# Autodesk Inventor assembly: 8 ball mechanism 3
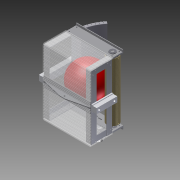
[picture p0: Inventor's stored thumbnail of the model, 180x180]
Saved by Autodesk Inventor 2012 (Build 160160000, 160)
## iProperties
Created: 2013-10-10
Part Number: 8 ball mechanism 3
Document SubType Name: Assembly
Designer: Bryce
Author: Bryce
## Documents named in this file (22)
- C:\Users\Bryce\Dropbox\Inventor Design Project Files\Independent Swerves\Inventor 2012\8 ball mechanism 3.iam
- C:\Users\Bryce\Dropbox\Inventor Design Project Files\Independent Swerves\Inventor 2012\8 ball corner L.ipt
- C:\Users\Bryce\Dropbox\Inventor Design Project Files\Independent Swerves\Inventor 2012\8 ball corner L_MIR.ipt
- C:\Users\Bryce\Dropbox\Inventor Design Project Files\Independent Swerves\Inventor 2012\8 ball polycarb side.ipt
- C:\Users\Bryce\Dropbox\Inventor Design Project Files\Independent Swerves\Inventor 2012\8 ball bottom 1 by 2 L short.ipt
- C:\Users\Bryce\Dropbox\Inventor Design Project Files\Independent Swerves\Inventor 2012\8 ball front L.ipt
- C:\Users\Bryce\Dropbox\Inventor Design Project Files\Independent Swerves\Inventor 2012\8 ball polycarb top 2.ipt
- C:\Users\Bryce\Dropbox\Inventor Design Project Files\Independent Swerves\Inventor 2012\8 ball bottom 1 by 2 L short_MIR.ipt
- C:\Users\Bryce\Dropbox\Inventor Design Project Files\Independent Swerves\Inventor 2012\8 ball corner L_MIR2.ipt
- C:\Users\Bryce\Dropbox\Inventor Design Project Files\Independent Swerves\Inventor 2012\8 ball corner L_MIR_MIR1.ipt
- C:\Users\Bryce\Dropbox\Inventor Design Project Files\Independent Swerves\Inventor 2012\8 ball polycarb side_MIR.ipt
- C:\Users\Bryce\Dropbox\Inventor Design Project Files\Independent Swerves\Inventor 2012\8 ball paint roller.ipt
- C:\Users\Bryce\Dropbox\Inventor Design Project Files\Independent Swerves\Inventor 2012\8 ball plastic slider.ipt
- C:\Users\Bryce\Dropbox\Inventor Design Project Files\Inventor library\Motors\Cimulator\CIMulator RS550 motor and 14T CIM gear assembly.iam
- C:\Users\Bryce\Dropbox\Inventor Design Project Files\Independent Swerves\Inventor 2012\8 ball ramp.ipt
- C:\Users\Bryce\Dropbox\Inventor Design Project Files\Independent Swerves\Inventor 2012\dodge ball.ipt
- C:\Users\Bryce\Dropbox\Inventor Design Project Files\Independent Swerves\Inventor 2012\8 ball top lift point.ipt
- C:\Users\Bryce\Dropbox\Inventor Design Project Files\Independent Swerves\Inventor 2012\8 ball top lift point_MIR.ipt
- C:\Users\Bryce\Dropbox\Inventor Design Project Files\Independent Swerves\Inventor 2012\8 ball plastic slider 2.ipt
- C:\Users\Bryce\Dropbox\Inventor Design Project Files\Inventor library\Bearings _ collars\Bearing flanged 1.125od .5id brf-06.ipt
- C:\Users\Bryce\Dropbox\Inventor Design Project Files\Independent Swerves\Inventor 2012\8 ball roller shaft.ipt
- C:\Users\Bryce\Dropbox\Inventor Design Project Files\Independent Swerves\Inventor 2012\8 ball roller plug.ipt
## Components (26 placed, 21 different names)
1. 8 ball bottom 1 by 2 L short:1 — Mate:1, Mate:2, Flush:1, Flush:2, Flush:3, Mate:10, Flush:11, Flush:11, Mate:32, Mate:35, Insert:2
2. 8 ball corner L:1 — Mate:1, Mate:2, Flush:1, Mate:14, Flush:13, Mate:15, Flush:15, Mate:48, Mate:62
3. 8 ball corner L_MIR:1 — Mate:10, Flush:11, Flush:11, Mate:31, Mate:33, Mate:34, Flush:31
4. 8 ball front L:1 — Mate:33, Mate:34, Mate:35
5. 8 ball front L:2 — Mate:66, Mate:67, Flush:31, Mate:68, Mate:69, Mate:70, Flush:32, Flush:33
6. 8 ball front L:3 — Mate:14, Flush:13, Mate:15, Flush:14, Flush:26, Mate:47, Mate:63
7. 8 ball polycarb top 2:1 — Flush:14, Flush:15, Flush:21, Flush:27, Flush:29, Mate:63, Mate:68
8. 8 ball polycarb side:2 — Mate:31, Mate:32, Flush:21, Flush:28
9. 8 ball bottom 1 by 2 L short_MIR:1 — Mate:36, Flush:22, Mate:37, Flush:23, Flush:24, Mate:38, Flush:25, Mate:39, Mate:40, Mate:42, Mate:45, Mate:50, Mate:55, Mate:56, Mate:57, Mate:58, Insert:1
10. 8 ball corner L_MIR2:1 — Mate:36, Flush:22, Mate:37, Mate:49, Mate:60
11. 8 ball corner L_MIR_MIR1:1 — Flush:24, Mate:38, Flush:25, Mate:41, Mate:66, Mate:67
12. 8 ball polycarb side_MIR:1 — Mate:40, Mate:41, Flush:26
13. 8 ball paint roller:1 — Mate:42, Mate:45, Mate:64, Insert:4, Insert:5, Mate:71
14. 8 ball plastic slider:1 — Flush:27, Flush:28, Flush:30, Mate:69
15. 8 ball plastic slider 2:1 — Mate:47, Flush:29, Flush:30
16. 8 ball front L:4 — Mate:48, Mate:49, Mate:50, Mate:59, Mate:61, Mate:62
17. CIMulator RS550 motor and 14T CIM gear assembly:1 [sub-assembly] — Mate:55, Mate:56, Mate:57, Mate:58
18. 8 ball ramp:1 — Mate:59, Mate:60, Mate:61, Mate:65
19. dodge ball:1 — Mate:64, Mate:65
20. 8 ball top lift point:1 — Mate:70, Flush:32, Flush:33
21. 8 ball top lift point_MIR:1
22. Bearing flanged 1.125od .5id brf-06:1 — Insert:1, Insert:3
23. Bearing flanged 1.125od .5id brf-06:2 — Insert:2
24. 8 ball roller shaft:1 — Insert:3, Flush:34, Flush:35
25. 8 ball roller plug:1 — Insert:4, Flush:35
26. 8 ball roller plug:2 — Insert:5, Flush:34, Mate:71
## Relationships (67: Mate 39, Flush 23, Insert 5)
- Mate:1: 8 ball bottom 1 by 2 L short:1 ↔ 8 ball corner L:1
- Mate:2: 8 ball bottom 1 by 2 L short:1 ↔ 8 ball corner L:1
- Flush:1: 8 ball bottom 1 by 2 L short:1 ↔ 8 ball corner L:1
- Flush:2 (-114.3 mm): 8 ball bottom 1 by 2 L short:1
- Flush:3 (152.4 mm): 8 ball bottom 1 by 2 L short:1
- Mate:10: 8 ball bottom 1 by 2 L short:1 ↔ 8 ball corner L_MIR:1
- Flush:11: 8 ball bottom 1 by 2 L short:1 ↔ 8 ball corner L_MIR:1
- Flush:11: 8 ball bottom 1 by 2 L short:1 ↔ 8 ball corner L_MIR:1
- Mate:14: 8 ball corner L:1 ↔ 8 ball front L:3
- Flush:13: 8 ball corner L:1 ↔ 8 ball front L:3
- Mate:15: 8 ball corner L:1 ↔ 8 ball front L:3
- Flush:14: 8 ball front L:3 ↔ 8 ball polycarb top 2:1
- Flush:15 (-0.254 mm): 8 ball corner L:1 ↔ 8 ball polycarb top 2:1
- Mate:31: 8 ball corner L_MIR:1 ↔ 8 ball polycarb side:2
- Mate:32: 8 ball bottom 1 by 2 L short:1 ↔ 8 ball polycarb side:2
- Flush:21: 8 ball polycarb top 2:1 ↔ 8 ball polycarb side:2
- Mate:33: 8 ball corner L_MIR:1 ↔ 8 ball front L:1
- Mate:34: 8 ball corner L_MIR:1 ↔ 8 ball front L:1
- Mate:35: 8 ball bottom 1 by 2 L short:1 ↔ 8 ball front L:1
- Mate:36: 8 ball bottom 1 by 2 L short_MIR:1 ↔ 8 ball corner L_MIR2:1
- Flush:22: 8 ball bottom 1 by 2 L short_MIR:1 ↔ 8 ball corner L_MIR2:1
- Mate:37: 8 ball bottom 1 by 2 L short_MIR:1 ↔ 8 ball corner L_MIR2:1
- Flush:23 (-114.3 mm): 8 ball bottom 1 by 2 L short_MIR:1
- Flush:24: 8 ball bottom 1 by 2 L short_MIR:1 ↔ 8 ball corner L_MIR_MIR1:1
- Mate:38: 8 ball bottom 1 by 2 L short_MIR:1 ↔ 8 ball corner L_MIR_MIR1:1
- Flush:25: 8 ball bottom 1 by 2 L short_MIR:1 ↔ 8 ball corner L_MIR_MIR1:1
- Mate:39 (152.4 mm): 8 ball bottom 1 by 2 L short_MIR:1
- Mate:40: 8 ball bottom 1 by 2 L short_MIR:1 ↔ 8 ball polycarb side_MIR:1
- Mate:41: 8 ball corner L_MIR_MIR1:1 ↔ 8 ball polycarb side_MIR:1
- Flush:26: 8 ball front L:3 ↔ 8 ball polycarb side_MIR:1
- Mate:42: 8 ball bottom 1 by 2 L short_MIR:1 ↔ 8 ball paint roller:1
- Mate:45 (19.05 mm): 8 ball bottom 1 by 2 L short_MIR:1 ↔ 8 ball paint roller:1
- Flush:27 (6.35 mm): 8 ball polycarb top 2:1 ↔ 8 ball plastic slider:1
- Flush:28 (142.875 mm): 8 ball polycarb side:2 ↔ 8 ball plastic slider:1
- Mate:47: 8 ball front L:3 ↔ 8 ball plastic slider 2:1
- Flush:29 (6.35 mm): 8 ball polycarb top 2:1 ↔ 8 ball plastic slider 2:1
- Flush:30: 8 ball plastic slider:1 ↔ 8 ball plastic slider 2:1
- Mate:48: 8 ball corner L:1 ↔ 8 ball front L:4
- Mate:49: 8 ball corner L_MIR2:1 ↔ 8 ball front L:4
- Mate:50: 8 ball bottom 1 by 2 L short_MIR:1 ↔ 8 ball front L:4
- Mate:55 (2.54 mm): 8 ball bottom 1 by 2 L short_MIR:1 ↔ CIMulator RS550 motor and 14T CIM gear assembly:1
- Mate:56 (2.54 mm): 8 ball bottom 1 by 2 L short_MIR:1 ↔ CIMulator RS550 motor and 14T CIM gear assembly:1
- Mate:57 (6.35 mm): 8 ball bottom 1 by 2 L short_MIR:1 ↔ CIMulator RS550 motor and 14T CIM gear assembly:1
- Mate:58: 8 ball bottom 1 by 2 L short_MIR:1 ↔ CIMulator RS550 motor and 14T CIM gear assembly:1
- Mate:59: 8 ball front L:4 ↔ 8 ball ramp:1
- Mate:60: 8 ball corner L_MIR2:1 ↔ 8 ball ramp:1
- Mate:61: 8 ball front L:4 ↔ 8 ball ramp:1
- Mate:62: 8 ball corner L:1 ↔ 8 ball front L:4
- Mate:63: 8 ball front L:3 ↔ 8 ball polycarb top 2:1
- Mate:64 (105.41 mm): 8 ball paint roller:1 ↔ dodge ball:1
- Mate:65 (80.01 mm): 8 ball ramp:1 ↔ dodge ball:1
- Mate:66: 8 ball front L:2 ↔ 8 ball corner L_MIR_MIR1:1
- Mate:67: 8 ball front L:2 ↔ 8 ball corner L_MIR_MIR1:1
- Flush:31: 8 ball corner L_MIR:1 ↔ 8 ball front L:2
- Mate:68: 8 ball front L:2 ↔ 8 ball polycarb top 2:1
- Mate:69: 8 ball front L:2 ↔ 8 ball plastic slider:1
- Mate:70: 8 ball front L:2 ↔ 8 ball top lift point:1
- Flush:32: 8 ball front L:2 ↔ 8 ball top lift point:1
- Flush:33 (127 mm): 8 ball front L:2 ↔ 8 ball top lift point:1
- Insert:1: 8 ball bottom 1 by 2 L short_MIR:1 ↔ Bearing flanged 1.125od .5id brf-06:1
- Insert:2: 8 ball bottom 1 by 2 L short:1 ↔ Bearing flanged 1.125od .5id brf-06:2
- Insert:3: Bearing flanged 1.125od .5id brf-06:1 ↔ 8 ball roller shaft:1
- Insert:4: 8 ball paint roller:1 ↔ 8 ball roller plug:1
- Insert:5: 8 ball paint roller:1 ↔ 8 ball roller plug:2
- Flush:34: 8 ball roller shaft:1 ↔ 8 ball roller plug:2
- Flush:35: 8 ball roller shaft:1 ↔ 8 ball roller plug:1
- Mate:71: 8 ball paint roller:1 ↔ 8 ball roller plug:2
